# Autodesk Inventor assembly: Mecanum_Assembly
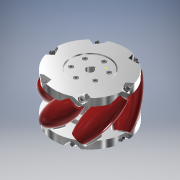
[picture p0: Inventor's stored thumbnail of the model, 180x180]
Saved by Autodesk Inventor 2018 (Build 220112000, 112)
## iProperties
Created: 2017-09-05
Part Number: Mecanum_Assembly
Document SubType Name: Assembly
Designer: P136265
Author: P136265
## Documents named in this file (11)
- C:\Users\P136265\Documents\mecanum-cad\Mecanum_Assembly.iam
- C:\Users\P136265\Documents\mecanum-cad\roller 8-19-6 bearing.ipt
- C:\Users\P136265\Documents\Inventor\Content Center Files\R2018\en-US\DIN 625 SKF(4)\DIN 625 SKF - SKF 619_8-2Z.ipt
- C:\Users\P136265\Documents\mecanum-cad\MecanumShaft.ipt
- C:\Users\P136265\Documents\mecanum-cad\PE_Sleeve.ipt
- C:\Users\P136265\Documents\mecanum-cad\CheekPlate.ipt
- C:\Users\P136265\Documents\mecanum-cad\MecanumHub.ipt
- C:\Users\P136265\Documents\mecanum-cad\Washer.ipt
- C:\Users\P136265\Documents\Inventor\Content Center Files\R2018\en-US\AS 1474(1)\AS 1474 - M8(1).ipt
- C:\Users\P136265\Documents\Inventor\Content Center Files\R2018\en-US\AS 1420\AS 1420 - 1973 - M6 x 30.ipt
- C:\Users\P136265\Documents\Inventor\Content Center Files\R2018\en-US\AS 1112 (2)\AS 1112 - M6  Type 5.ipt
## Components (81 placed, 10 different names)
1. CheekPlate:1 — Mate:11, Mate:12, Mate:13, Angle:3, Mate:18, Mate:19, Mate:21, Mate:24, Mate:25
2. CheekPlate:2 — Angle:3, Mate:14, Mate:15, Mate:23, Mate:28, Mate:29
3. MecanumHub:1 — Mate:18, Mate:19, Mate:27, Mate:31
4. roller 8-19-6 bearing:1 — Mate:1, Angle:1, Mate:2, Mate:3, Mate:4, Insert:1, Insert:2, Angle:2, Mate:9, Mate:15
5. MecanumShaft:1 — Angle:2, Mate:9, Mate:10, Mate:20, Mate:22
6. PE_Sleeve:1 — Mate:3, Mate:4
7. Washer:1 — Mate:5, Mate:6
8. Washer:2 — Mate:7, Mate:8, Mate:10
9. DIN 625 SKF- with two Z shields SKF 619/8-2Z:1 — Insert:1, Mate:7, Mate:8
10. DIN 625 SKF- with two Z shields SKF 619/8-2Z:2 — Insert:2, Mate:5, Mate:6
11. roller 8-19-6 bearing:2
12. MecanumShaft:2
13. PE_Sleeve:2
14. Washer:3
15. Washer:4
16. DIN 625 SKF- with two Z shields SKF 619/8-2Z:3
17. DIN 625 SKF- with two Z shields SKF 619/8-2Z:4
18. roller 8-19-6 bearing:3
19. MecanumShaft:3 — Mate:11
20. PE_Sleeve:3
21. Washer:5 — Mate:12
22. Washer:6
23. DIN 625 SKF- with two Z shields SKF 619/8-2Z:5
24. DIN 625 SKF- with two Z shields SKF 619/8-2Z:6
25. roller 8-19-6 bearing:4
26. MecanumShaft:4 — Mate:14
27. PE_Sleeve:4
28. Washer:7
29. Washer:8
30. DIN 625 SKF- with two Z shields SKF 619/8-2Z:7
31. DIN 625 SKF- with two Z shields SKF 619/8-2Z:8
32. roller 8-19-6 bearing:5 — Mate:13
33. MecanumShaft:5
34. PE_Sleeve:5
35. Washer:9
36. Washer:10
37. DIN 625 SKF- with two Z shields SKF 619/8-2Z:9
38. DIN 625 SKF- with two Z shields SKF 619/8-2Z:10
39. roller 8-19-6 bearing:6
40. MecanumShaft:6
41. PE_Sleeve:6
42. Washer:11
43. Washer:12
44. DIN 625 SKF- with two Z shields SKF 619/8-2Z:11
45. DIN 625 SKF- with two Z shields SKF 619/8-2Z:12
46. AS 1474 - Metric M8:1 — Mate:20, Mate:21
47. AS 1474 - Metric M8:2 — Mate:22, Mate:23
48. AS 1474 - Metric M8:3
49. AS 1474 - Metric M8:4
50. AS 1474 - Metric M8:5
51. AS 1474 - Metric M8:6
52. AS 1474 - Metric M8:7
53. AS 1474 - Metric M8:8
54. AS 1474 - Metric M8:9
55. AS 1474 - Metric M8:10
56. AS 1474 - Metric M8:11
57. AS 1474 - Metric M8:12
58. AS 1420 - Metric M6 x 30:1 — Mate:24, Mate:25, Mate:26
59. AS 1420 - Metric M6 x 30:2
60. AS 1420 - Metric M6 x 30:3
61. AS 1420 - Metric M6 x 30:4
62. AS 1420 - Metric M6 x 30:5
63. AS 1420 - Metric M6 x 30:6
64. AS 1112 (2) - Metric M6  Type 5:1 — Mate:26, Mate:27
65. AS 1112 (2) - Metric M6  Type 5:2
66. AS 1112 (2) - Metric M6  Type 5:3
67. AS 1112 (2) - Metric M6  Type 5:4
68. AS 1112 (2) - Metric M6  Type 5:5
69. AS 1112 (2) - Metric M6  Type 5:6
70. AS 1420 - Metric M6 x 30:7 — Mate:28, Mate:29, Mate:30
71. AS 1420 - Metric M6 x 30:8
72. AS 1420 - Metric M6 x 30:9
73. AS 1420 - Metric M6 x 30:10
74. AS 1420 - Metric M6 x 30:11
75. AS 1420 - Metric M6 x 30:12
76. AS 1112 (2) - Metric M6  Type 5:7 — Mate:30, Mate:31
77. AS 1112 (2) - Metric M6  Type 5:8
78. AS 1112 (2) - Metric M6  Type 5:9
79. AS 1112 (2) - Metric M6  Type 5:10
80. AS 1112 (2) - Metric M6  Type 5:11
81. AS 1112 (2) - Metric M6  Type 5:12
## Component patterns: (6 elements, first: roller 8-19-6 bearing:1 + MecanumShaft:1 + PE_Sleeve:1 + Washer:1 + Washer:2 + DIN 625 SKF- with two Z shields SKF 619/8-2Z:1 + DIN 625 SKF- with two Z shields SKF 619/8-2Z:2), (6 elements, first: AS 1474 - Metric M8:1 + AS 1474 - Metric M8:2), (6 elements, first: AS 1420 - Metric M6 x 30:1), (6 elements, first: AS 1112 (2) - Metric M6  Type 5:1), (6 elements, first: AS 1420 - Metric M6 x 30:7), (6 elements, first: AS 1112 (2) - Metric M6  Type 5:7)
## Relationships (34: Mate 29, Angle 3, Insert 2)
- Mate:1 (75 mm): roller 8-19-6 bearing:1
- Angle:1 (45 deg): roller 8-19-6 bearing:1
- Mate:2: roller 8-19-6 bearing:1
- Mate:3: roller 8-19-6 bearing:1 ↔ PE_Sleeve:1
- Mate:4: roller 8-19-6 bearing:1 ↔ PE_Sleeve:1
- Insert:1: roller 8-19-6 bearing:1 ↔ DIN 625 SKF- with two Z shields SKF 619/8-2Z:1
- Insert:2: roller 8-19-6 bearing:1 ↔ DIN 625 SKF- with two Z shields SKF 619/8-2Z:2
- Mate:5: Washer:1 ↔ DIN 625 SKF- with two Z shields SKF 619/8-2Z:2
- Mate:6: Washer:1 ↔ DIN 625 SKF- with two Z shields SKF 619/8-2Z:2
- Mate:7: Washer:2 ↔ DIN 625 SKF- with two Z shields SKF 619/8-2Z:1
- Mate:8: Washer:2 ↔ DIN 625 SKF- with two Z shields SKF 619/8-2Z:1
- Angle:2 (0 deg): roller 8-19-6 bearing:1 ↔ MecanumShaft:1
- Mate:9: roller 8-19-6 bearing:1 ↔ MecanumShaft:1
- Mate:10 (18 mm): MecanumShaft:1 ↔ Washer:2
- Mate:11: CheekPlate:1 ↔ MecanumShaft:3
- Mate:12: CheekPlate:1 ↔ Washer:5
- Mate:13: CheekPlate:1 ↔ roller 8-19-6 bearing:5
- Angle:3 (0 deg): CheekPlate:1 ↔ CheekPlate:2
- Mate:14: CheekPlate:2 ↔ MecanumShaft:4
- Mate:15: CheekPlate:2 ↔ roller 8-19-6 bearing:1
- Mate:18: CheekPlate:1 ↔ MecanumHub:1
- Mate:19: CheekPlate:1 ↔ MecanumHub:1
- Mate:20: MecanumShaft:1 ↔ AS 1474 - Metric M8:1
- Mate:21: CheekPlate:1 ↔ AS 1474 - Metric M8:1
- Mate:22: MecanumShaft:1 ↔ AS 1474 - Metric M8:2
- Mate:23: CheekPlate:2 ↔ AS 1474 - Metric M8:2
- Mate:24: CheekPlate:1 ↔ AS 1420 - Metric M6 x 30:1
- Mate:25: CheekPlate:1 ↔ AS 1420 - Metric M6 x 30:1
- Mate:26: AS 1420 - Metric M6 x 30:1 ↔ AS 1112 (2) - Metric M6  Type 5:1
- Mate:27: MecanumHub:1 ↔ AS 1112 (2) - Metric M6  Type 5:1
- Mate:28: CheekPlate:2 ↔ AS 1420 - Metric M6 x 30:7
- Mate:29: CheekPlate:2 ↔ AS 1420 - Metric M6 x 30:7
- Mate:30: AS 1420 - Metric M6 x 30:7 ↔ AS 1112 (2) - Metric M6  Type 5:7
- Mate:31: MecanumHub:1 ↔ AS 1112 (2) - Metric M6  Type 5:7
